# Autodesk Inventor assembly: assbemle
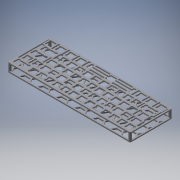
[picture p0: Inventor's stored thumbnail of the model, 180x180]
Saved by Autodesk Inventor 2019 (Build 230136000, 136)
## iProperties
Created: 2019-01-24
Part Number: assbemle
Document SubType Name: Assembly
Designer: Andrew
Author: Andrew
## Documents named in this file (4)
- C:\Users\Andrew\Desktop\assbemle.iam
- C:\Users\Andrew\Desktop\BottomPlate.ipt
- C:\Users\Andrew\Desktop\Pillar.ipt
- C:\Users\Andrew\Desktop\TopPlate.ipt
## Components (6 placed, 3 different names)
1. BottomPlate:1 — Rotational:1, Rotational:2, Rotational:3, Rotational:4
2. Pillar:1 — Rotational:1
3. Pillar:2 — Rotational:2, Cylindrical:1
4. Pillar:3 — Rotational:4
5. Pillar:4 — Rotational:3, Rotational:5
6. TopPlate:1 — Rotational:5, Cylindrical:1
## Relationships (6: RevoluteJoint 5, CylindricalJoint 1)
- Rotational:1 [RevoluteJoint]: BottomPlate:1 ↔ Pillar:1
- Rotational:2 [RevoluteJoint]: BottomPlate:1 ↔ Pillar:2
- Rotational:3 [RevoluteJoint]: BottomPlate:1 ↔ Pillar:4
- Rotational:4 [RevoluteJoint]: BottomPlate:1 ↔ Pillar:3
- Rotational:5 [RevoluteJoint]: Pillar:4 ↔ TopPlate:1
- Cylindrical:1: Pillar:2 ↔ TopPlate:1
